# Autodesk Inventor assembly: Electrical Board - front top
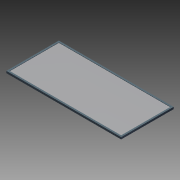
[picture p0: Inventor's stored thumbnail of the model, 180x180]
Saved by Autodesk Inventor 2012 (Build 160160000, 160)
## iProperties
Created: 2012-01-14
Part Number: Electrical Board - front top
Document SubType Name: Assembly
Designer: Antonella Wilby
Author: Antonella Wilby
## Documents named in this file (4)
- C:\Users\Antonella\Documents\GCC Robotics 2012 - Mechanical\Robot 2.0\Electrical\Front Electrical Board\Top\Electrical Board - front top.iam
- C:\Users\Antonella\Documents\GCC Robotics 2012 - Mechanical\Robot 2.0\Electrical\Front Electrical Board\Top\Electrical Board - front top.ipt
- C:\Users\Antonella\Documents\GCC Robotics 2012 - Mechanical\Robot 2.0\Electrical\Front Electrical Board\Top\frame long.ipt
- C:\Users\Antonella\Documents\GCC Robotics 2012 - Mechanical\Robot 2.0\Electrical\Front Electrical Board\Top\frame short.ipt
## Components (5 placed, 3 different names)
1. Electrical Board - front top:1 — Mate:1, Flush:2, Mate:2, Mate:3, Mate:4, Mate:5, Mate:6, Mate:7, Mate:8, Mate:9, Mate:10, Flush:3
2. frame long:1 — Mate:1, Flush:2, Mate:2
3. frame long:2 — Mate:6, Mate:7, Mate:8
4. frame short:1 — Mate:3, Mate:4, Mate:5
5. frame short:2 — Mate:9, Mate:10, Flush:3
## Relationships (12: Mate 10, Flush 2)
- Mate:1: Electrical Board - front top:1 ↔ frame long:1
- Flush:2: Electrical Board - front top:1 ↔ frame long:1
- Mate:2: Electrical Board - front top:1 ↔ frame long:1
- Mate:3: Electrical Board - front top:1 ↔ frame short:1
- Mate:4: Electrical Board - front top:1 ↔ frame short:1
- Mate:5: Electrical Board - front top:1 ↔ frame short:1
- Mate:6: Electrical Board - front top:1 ↔ frame long:2
- Mate:7: Electrical Board - front top:1 ↔ frame long:2
- Mate:8: Electrical Board - front top:1 ↔ frame long:2
- Mate:9: Electrical Board - front top:1 ↔ frame short:2
- Mate:10: Electrical Board - front top:1 ↔ frame short:2
- Flush:3: Electrical Board - front top:1 ↔ frame short:2
